# Autodesk Inventor assembly: 3_CIM_Ball_Shifter_Base_Kit_with_3rd_Stage_217-3268
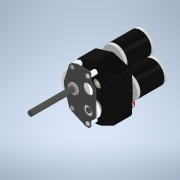
[picture p0: Inventor's stored thumbnail of the model, 180x180]
Saved by Autodesk Inventor 2020 (Build 240168000, 168)
## iProperties
Created: 2015-12-17
Part Number: 3_CIM_Ball_Shifter_Base_Kit_with_3rd_Stage_217-3268
Description: STEP AP214
Document SubType Name: Assembly
Designer: srini
Sending System: SolidWorks 2015
Preprocessor: SwSTEP 2.0
Title: 217-3268-STEP-20151217.STEP
Revision Number: ANY
## Documents named in this file (56)
- C:\Users\srini\Documents\FRC\2020\SuperShifter\3_CIM_Ball_Shifter_Base_Kit_with_3rd_Stage_217-3268.iam
- C:\Users\srini\Documents\FRC\2020\SuperShifter\217-2733-001 Rev2.ipt
- C:\Users\srini\Documents\FRC\2020\SuperShifter\217-2731-001 Rev2.ipt
- C:\Users\srini\Documents\FRC\2020\SuperShifter\217-2789-001 Rev2.ipt
- C:\Users\srini\Documents\FRC\2020\SuperShifter\217-2778-001 Rev2_NCQ8A075-050M.iam
- C:\Users\srini\Documents\FRC\2020\SuperShifter\217-2428-012 Rev2.ipt
- C:\Users\srini\Documents\FRC\2020\SuperShifter\217-2428-005 Rev1.ipt
- C:\Users\srini\Documents\FRC\2020\SuperShifter\SCREW-832-0375.ipt
- C:\Users\srini\Documents\FRC\2020\SuperShifter\SBS1_SBS-0632-0250.ipt
- C:\Users\srini\Documents\FRC\2020\SuperShifter\217-4098-100 Rev1.iam
- C:\Users\srini\Documents\FRC\2020\SuperShifter\217-2428-017 Rev2.ipt
- C:\Users\srini\Documents\FRC\2020\SuperShifter\217-2428-016 Rev3_Spur01.ipt
- C:\Users\srini\Documents\FRC\2020\SuperShifter\217-2428-019 Rev1.ipt
- C:\Users\srini\Documents\FRC\2020\SuperShifter\217-2428-006 Rev1.ipt
- C:\Users\srini\Documents\FRC\2020\SuperShifter\217-2614-001_12t.ipt
- C:\Users\srini\Documents\FRC\2020\SuperShifter\217-2761-001 rev1.ipt
- C:\Users\srini\Documents\FRC\2020\SuperShifter\217-3195-002 rev2.ipt
- C:\Users\srini\Documents\FRC\2020\SuperShifter\217-3195-001 Rev1.ipt
- C:\Users\srini\Documents\FRC\2020\SuperShifter\276-1027-001.ipt
- C:\Users\srini\Documents\FRC\2020\SuperShifter\SCREW-832-1750.ipt
- C:\Users\srini\Documents\FRC\2020\SuperShifter\217-2428-004 Rev3.ipt
- C:\Users\srini\Documents\FRC\2020\SuperShifter\217-2428-021 Rev1.ipt
- C:\Users\srini\Documents\FRC\2020\SuperShifter\217-2428-029 Rev1.ipt
- C:\Users\srini\Documents\FRC\2020\SuperShifter\Grayhill Lock Washer.ipt
- C:\Users\srini\Documents\FRC\2020\SuperShifter\Grayhill Nut.ipt
- C:\Users\srini\Documents\FRC\2020\SuperShifter\Grahill Encoder.ipt
- C:\Users\srini\Documents\FRC\2020\SuperShifter\SBS1_SBS-2520-125.ipt
- C:\Users\srini\Documents\FRC\2020\SuperShifter\217-3195-008 Rev1_stubby .75_.ipt
- C:\Users\srini\Documents\FRC\2020\SuperShifter\Nylock Nut_NNY2520-ZC.ipt
- C:\Users\srini\Documents\FRC\2020\SuperShifter\SBS1_SBS2520-0625ZC.ipt
- C:\Users\srini\Documents\FRC\2020\SuperShifter\217-2617-002 Rev1_91780A359.ipt
- C:\Users\srini\Documents\FRC\2020\SuperShifter\217-3195-003 rev2.ipt
- C:\Users\srini\Documents\FRC\2020\SuperShifter\217-2617-003 Rev1.ipt
- C:\Users\srini\Documents\FRC\2020\SuperShifter\217-3109-001 Rev1.ipt
- C:\Users\srini\Documents\FRC\2020\SuperShifter\217-2734-001 Rev3.ipt
- C:\Users\srini\Documents\FRC\2020\SuperShifter\217-2617-004 Rev1_97431A340_grv.ipt
- C:\Users\srini\Documents\FRC\2020\SuperShifter\217-2702-001_20t.ipt
- C:\Users\srini\Documents\FRC\2020\SuperShifter\217-2715-002 Rev1_64t.ipt
- C:\Users\srini\Documents\FRC\2020\SuperShifter\217-2704-001_24.ipt
- C:\Users\srini\Documents\FRC\2020\SuperShifter\217-2714-002 Rev1_60t.ipt
- C:\Users\srini\Documents\FRC\2020\SuperShifter\217-3221-002 Rev1.ipt
- C:\Users\srini\Documents\FRC\2020\SuperShifter\217-2705-001_30t.ipt
- C:\Users\srini\Documents\FRC\2020\SuperShifter\217-2712-002 Rev1_50t.ipt
- C:\Users\srini\Documents\FRC\2020\SuperShifter\217-2706-001_34t.ipt
- C:\Users\srini\Documents\FRC\2020\SuperShifter\217-3287-001 Rev3.iam
- C:\Users\srini\Documents\FRC\2020\SuperShifter\217-3211-001 Rev1_34t.ipt
- C:\Users\srini\Documents\FRC\2020\SuperShifter\217-3288-001 Rev3.iam
- C:\Users\srini\Documents\FRC\2020\SuperShifter\217-3210-001 Rev1_30t.ipt
- C:\Users\srini\Documents\FRC\2020\SuperShifter\217-3292-001 Rev3.iam
- C:\Users\srini\Documents\FRC\2020\SuperShifter\217-2703-001.ipt
- C:\Users\srini\Documents\FRC\2020\SuperShifter\217-2711-002 Rev1_50t.ipt
- C:\Users\srini\Documents\FRC\2020\SuperShifter\217-2428-023 Rev1_9714K3.ipt
- C:\Users\srini\Documents\FRC\2020\SuperShifter\SBS_SBS2520-1750.ipt
- C:\Users\srini\Documents\FRC\2020\SuperShifter\NNYXXXX-ZZ_NNY2520-ZC.ipt
- C:\Users\srini\Documents\FRC\2020\SuperShifter\SBS_SBS2520-1500ZC.ipt
- C:\Users\srini\Documents\FRC\2020\SuperShifter\Mini_CIM_Motor_217-3371.ipt
## Components (83 placed, 81 different names)
1. 217-2733-001 Rev2_1
2. 217-2733-001 Rev2_2
3. 217-2731-001 Rev2_3
4. 217-2789-001 Rev2_4
5. 217-2778-001 Rev2_NCQ8A075-050M_5 [sub-assembly]
6. 217-2428-012 Rev2_6
7. 217-2428-005 Rev1_7
8. 217-2428-005 Rev1_8
9. SCREW-832-0375_9
10. SCREW-832-0375_10
11. SCREW-832-0375_11
12. SCREW-832-0375_12
13. SBS1_SBS-0632-0250_13
14. SBS1_SBS-0632-0250_14
15. 217-4098-100 Rev1_15 [sub-assembly]
16. 217-2428-017 Rev2_16
17. 217-2428-016 Rev3_Spur01_17
18. 217-2428-019 Rev1_18
19. 217-2428-006 Rev1_19
20. 217-2428-006 Rev1_20
21. SCREW-832-0375_21
22. SCREW-832-0375_22
23. SCREW-832-0375_23
24. SCREW-832-0375_24
25. 217-2614-001_12t_25
26. 217-2761-001 rev1_26
27. 217-2761-001 rev1_27
28. 217-2614-001_12t_28
29. 217-2614-001_12t_29
30. 217-2761-001 rev1_30
31. 217-3195-002 rev2_31
32. 217-3195-001 Rev1_32 — Insert:1, Insert:2, Insert:3, Insert:4, Insert:5, Insert:6
33. 276-1027-001_33
34. 276-1027-001_34
35. SCREW-832-1750_35
36. SCREW-832-1750_36
37. 217-2428-004 Rev3_37
38. 217-2428-021 Rev1_38
39. 217-2428-029 Rev1_39
40. Grayhill Lock Washer_40
41. Grayhill Nut_41
42. Grahill Encoder_45
43. SBS1_SBS-2520-125_46
44. 217-3195-008 Rev1_stubby .75"_47
45. 217-3195-008 Rev1_stubby .75"_48
46. Nylock Nut_NNY2520-ZC_49
47. Nylock Nut_NNY2520-ZC_50
48. SBS1_SBS2520-0625ZC_51
49. SBS1_SBS2520-0625ZC_52
50. 217-2617-002 Rev1_91780A359_53
51. 217-2617-002 Rev1_91780A359_54
52. 217-3195-003 rev2_55
53. 217-2617-003 Rev1_56
54. 217-3109-001 Rev1_57
55. 217-2734-001 Rev3_58
56. 217-2617-004 Rev1_97431A340_grv_59
57. 217-2617-004 Rev1_97431A340_grv_60
58. 217-2702-001_20t_61
59. 217-2715-002 Rev1_64t_62
60. 217-2704-001_24_63
61. 217-2714-002 Rev1_60t_64
62. 217-3221-002 Rev1_65
63. 217-2705-001_30t_66
64. 217-2712-002 Rev1_50t_67
65. 217-2706-001_34t_68
66. SBS1_SBS-2520-125_69
67. 217-3287-001 Rev3_70 [sub-assembly]
68. 217-3211-001 Rev1_34t_71
69. 217-3288-001 Rev3_72 [sub-assembly]
70. 217-3210-001 Rev1_30t_73
71. 217-3292-001 Rev3_74 [sub-assembly]
72. 217-2703-001_75
73. 217-2711-002 Rev1_50t_76
74. 217-2428-023 Rev1_9714K3_77
75. SBS_SBS2520-1750_78
76. SBS_SBS2520-1750_79
77. NNYXXXX-ZZ_NNY2520-ZC_80
78. NNYXXXX-ZZ_NNY2520-ZC_81
79. SBS_SBS2520-1500ZC_82
80. SBS_SBS2520-1500ZC_83
81. Mini_CIM_Motor_217-3371:1 — Insert:3, Insert:4
82. Mini_CIM_Motor_217-3371:2 — Insert:1, Insert:2
83. Mini_CIM_Motor_217-3371:3 — Insert:5, Insert:6
## Relationships (6: Insert 6)
- Insert:1: 217-3195-001 Rev1_32 ↔ Mini_CIM_Motor_217-3371:2
- Insert:2: 217-3195-001 Rev1_32 ↔ Mini_CIM_Motor_217-3371:2
- Insert:3: 217-3195-001 Rev1_32 ↔ Mini_CIM_Motor_217-3371:1
- Insert:4: 217-3195-001 Rev1_32 ↔ Mini_CIM_Motor_217-3371:1
- Insert:5: 217-3195-001 Rev1_32 ↔ Mini_CIM_Motor_217-3371:3
- Insert:6: 217-3195-001 Rev1_32 ↔ Mini_CIM_Motor_217-3371:3
